# Autodesk Inventor assembly: cadeiraEgarfo
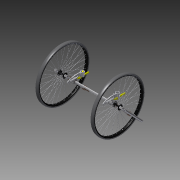
[picture p0: Inventor's stored thumbnail of the model, 180x180]
Saved by Autodesk Inventor 2015 (Build 190159000, 159)
## iProperties
Created: 2016-08-11
Part Number: cadeiraEgarfo
Document SubType Name: Assembly
Designer: EriveltonDell
Author: EriveltonDell
## Documents named in this file (8)
- C:\Users\EriveltonDell\Documents\Centro Universitário da FEI\Wheelchair\CADEIRA DE RODAS - DESENHO\Model\cadeiraEgarfo.iam
- C:\Users\EriveltonDell\Documents\Centro Universitário da FEI\Wheelchair\CADEIRA DE RODAS - DESENHO\Model\Koło_tylne.iam
- C:\Users\EriveltonDell\Documents\Centro Universitário da FEI\Wheelchair\CADEIRA DE RODAS - DESENHO\Model\GARFO.ipt
- C:\Users\EriveltonDell\Documents\Centro Universitário da FEI\Wheelchair\CADEIRA DE RODAS - DESENHO\Model\suporte-barra.ipt
- C:\Users\EriveltonDell\Documents\Centro Universitário da FEI\Wheelchair\CADEIRA DE RODAS - DESENHO\Model\Barra-garfo.ipt
- C:\Users\EriveltonDell\Documents\Centro Universitário da FEI\Wheelchair\CADEIRA DE RODAS - DESENHO\Model\suporte-rodas.ipt
- C:\Users\EriveltonDell\Documents\Centro Universitário da FEI\Wheelchair\CADEIRA DE RODAS - DESENHO\Model\suporte-rodas-esq.ipt
- C:\Users\EriveltonDell\Documents\Centro Universitário da FEI\Wheelchair\CADEIRA DE RODAS - DESENHO\Model\suporte-eixo-new.ipt
## Components (14 placed, 7 different names)
1. Koło_tylne:1 [sub-assembly] — Tangent:5, Angle:5
2. Koło_tylne:2 [sub-assembly] — Tangent:5
3. GARFO:1 — Tangent:8
4. GARFO:2 — Insert:3, Angle:4
5. suporte-barra:1 — Mate:4, Tangent:4
6. suporte-barra:2
7. Barra-garfo:1 — Mate:4, Tangent:4
8. suporte-barra:3 — Tangent:8, Insert:5
9. suporte-barra:4 — Insert:3, Insert:4
10. Barra-garfo:2
11. suporte-rodas:1 — Mate:7, Tangent:9, Tangent:10, Angle:3, Angle:4
12. suporte-rodas-esq:1 — Mate:8, Tangent:11, Tangent:12, Angle:3, Angle:5
13. suporte-eixo-new:1 — Insert:4, Mate:7, Tangent:9, Tangent:10
14. suporte-eixo-new:2 — Insert:5, Mate:8, Tangent:11, Tangent:12
## Relationships (30: Tangent 12, Mate 8, Insert 5, Angle 5)
- [Mate]: Koło_tylne:1 ↔ GARFO:1
- [Tangent]: Koło_tylne:1 ↔ GARFO:1
- [Tangent]: Koło_tylne:2 ↔ GARFO:2
- [Mate]: Koło_tylne:2 ↔ GARFO:2
- [Insert]: GARFO:1 ↔ suporte-barra:1
- [Angle] (0 deg): Koło_tylne:1 ↔ suporte-barra:1
- [Insert]: GARFO:2 ↔ suporte-barra:2
- [Angle] (0 deg): GARFO:2 ↔ suporte-barra:2
- [Mate]: suporte-barra:2 ↔ Barra-garfo:1
- [Tangent]: suporte-barra:2 ↔ Barra-garfo:1
- Mate:4: suporte-barra:1 ↔ Barra-garfo:1
- Tangent:4: suporte-barra:1 ↔ Barra-garfo:1
- Tangent:5: Koło_tylne:1 ↔ Koło_tylne:2
- [Mate]: suporte-barra:4 ↔ Barra-garfo:2
- [Tangent]: suporte-barra:4 ↔ Barra-garfo:2
- [Mate]: suporte-barra:3 ↔ Barra-garfo:2
- [Tangent]: suporte-barra:3 ↔ Barra-garfo:2
- Insert:3 (-100 mm): GARFO:2 ↔ suporte-barra:4
- Tangent:8: GARFO:1 ↔ suporte-barra:3
- Insert:4: suporte-barra:4 ↔ suporte-eixo-new:1
- Insert:5 (-25.4 mm): suporte-barra:3 ↔ suporte-eixo-new:2
- Mate:7: suporte-rodas:1 ↔ suporte-eixo-new:1
- Tangent:9: suporte-rodas:1 ↔ suporte-eixo-new:1
- Tangent:10: suporte-rodas:1 ↔ suporte-eixo-new:1
- Mate:8: suporte-rodas-esq:1 ↔ suporte-eixo-new:2
- Tangent:11: suporte-rodas-esq:1 ↔ suporte-eixo-new:2
- Tangent:12: suporte-rodas-esq:1 ↔ suporte-eixo-new:2
- Angle:3 (0 deg): suporte-rodas:1 ↔ suporte-rodas-esq:1
- Angle:4 (45 deg): GARFO:2 ↔ suporte-rodas:1
- Angle:5 (0 deg): Koło_tylne:1 ↔ suporte-rodas-esq:1
## Named parameters: d13_d10 = 0 mm, d14_d11 = 0 mm, d15_d98 = 0 mm, d16_d99 = 0 mm, sa_0 = 4.5e-11, sa_1 = -34991.3, sa_2 = 779.219
note: some values were not read from the file. Shown as the stored number, unit unknown: "sa_0", "sa_1", "sa_2".
